# Autodesk Inventor assembly: base_body
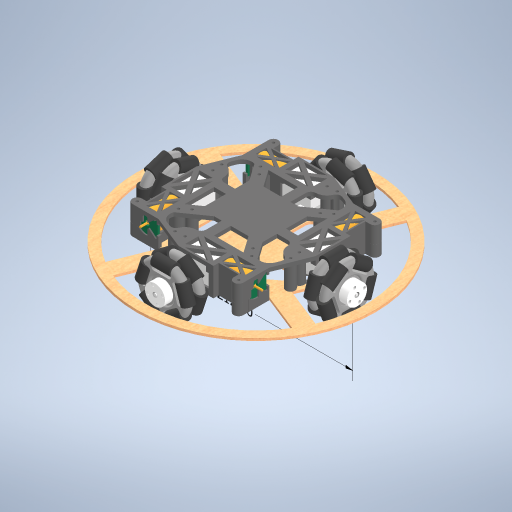
[picture p0: Inventor's stored thumbnail of the model, 512x512]
Saved by Autodesk Inventor 2024.1 (Build 281209000, 209)
## iProperties
Created: 2024-07-01
Part Number: base_body
Document SubType Name: Assembly
Designer: hibik
Author: hibik
## Documents named in this file (8)
- C:\Users\hibik\Desktop\ロボメカ\Rescue\2年\子機_本選\base_body.iam
- C:\Users\hibik\Desktop\ロボメカ\Rescue\2年\子機_本選\body_upper.ipt
- C:\Users\hibik\Desktop\ロボメカ\Rescue\2年\子機_本選\Motor.ipt
- C:\Users\hibik\Desktop\ロボメカ\Rescue\2年\子機_本選\encoder.ipt
- C:\Users\hibik\Desktop\ロボメカ\Rescue\2年\子機_本選\Motor_400.ipt
- C:\Users\hibik\Desktop\ロボメカ\Rescue\2年\子機_本選\オムニホイール.iam
- C:\Users\hibik\Desktop\ロボメカ\Rescue\2年\子機_本選\body_under.ipt
- C:\Users\hibik\Desktop\ロボメカ\Rescue\2年\子機_本選\plate.ipt
## Components (22 placed, 7 different names)
1. body_upper:1 — メイト:1, メイト:2, メイト:3, メイト:4, メイト:5, メイト:6, メイト:7, メイト:8, メイト:9, メイト:10, メイト:11, メイト:12, 挿入:1, 挿入:2, 挿入:3, 挿入:4, 角度:1, 角度:2, 角度:3, 角度:4, 挿入:5, 角度:5, 挿入:6, 角度:6, 挿入:7, 角度:7, 挿入:8, 角度:8, メイト:13, メイト:14, メイト:15, メイト:16, メイト:17, フラッシュ:1, フラッシュ:2
2. Motor:1 — メイト:1, メイト:9, メイト:10, 回転:1
3. Motor:2 — メイト:2, メイト:7, メイト:8, 回転:4
4. Motor:3 — メイト:4, メイト:5, メイト:6, 回転:3
5. Motor:4 — メイト:3, メイト:11, メイト:12, 回転:2
6. encoder:1 — 挿入:1, 角度:2
7. encoder:2 — 挿入:4, 角度:1
8. encoder:3 — 挿入:3, 角度:4
9. encoder:4 — 挿入:2, 角度:3
10. Motor_400:1 — 挿入:5, 角度:5, 挿入:11
11. Motor_400:2 — 挿入:6, 角度:6, 挿入:12
12. Motor_400:3 — 挿入:7, 角度:7, 挿入:9
13. Motor_400:4 — 挿入:8, 角度:8, 挿入:10
14. オムニホイール:1 [sub-assembly] — 回転:3
15. オムニホイール:2 [sub-assembly] — 回転:4
16. オムニホイール:3 [sub-assembly] — 回転:2
17. オムニホイール:4 [sub-assembly] — 回転:1
18. body_under:1 — 挿入:9, メイト:13
19. body_under:2 — 挿入:12, メイト:16
20. body_under:3 — 挿入:11, メイト:15
21. body_under:4 — 挿入:10, メイト:14
22. plate:1 — メイト:17, フラッシュ:1, フラッシュ:2
## Relationships (43: Mate 17, Insert 12, Angle 8, RevoluteJoint 4, Flush 2)
- メイト:1 [Mate]: body_upper:1 ↔ Motor:1
- メイト:2 [Mate]: body_upper:1 ↔ Motor:2
- メイト:3 [Mate]: body_upper:1 ↔ Motor:4
- メイト:4 [Mate]: body_upper:1 ↔ Motor:3
- メイト:5 [Mate]: body_upper:1 ↔ Motor:3
- メイト:6 [Mate]: body_upper:1 ↔ Motor:3
- メイト:7 [Mate]: body_upper:1 ↔ Motor:2
- メイト:8 [Mate]: body_upper:1 ↔ Motor:2
- メイト:9 [Mate]: body_upper:1 ↔ Motor:1
- メイト:10 [Mate]: body_upper:1 ↔ Motor:1
- メイト:11 [Mate]: body_upper:1 ↔ Motor:4
- メイト:12 [Mate]: body_upper:1 ↔ Motor:4
- 挿入:1 [Insert]: body_upper:1 ↔ encoder:1
- 挿入:2 [Insert]: body_upper:1 ↔ encoder:4
- 挿入:3 [Insert]: body_upper:1 ↔ encoder:3
- 挿入:4 [Insert]: body_upper:1 ↔ encoder:2
- 角度:1 [Angle] (0 deg): body_upper:1 ↔ encoder:2
- 角度:2 [Angle] (0 deg): body_upper:1 ↔ encoder:1
- 角度:3 [Angle] (0 deg): body_upper:1 ↔ encoder:4
- 角度:4 [Angle] (0 deg): body_upper:1 ↔ encoder:3
- 挿入:5 [Insert]: body_upper:1 ↔ Motor_400:1
- 角度:5 [Angle] (0 deg): body_upper:1 ↔ Motor_400:1
- 挿入:6 [Insert]: body_upper:1 ↔ Motor_400:2
- 角度:6 [Angle] (0 deg): body_upper:1 ↔ Motor_400:2
- 挿入:7 [Insert]: body_upper:1 ↔ Motor_400:3
- 角度:7 [Angle] (0 deg): body_upper:1 ↔ Motor_400:3
- 挿入:8 [Insert]: body_upper:1 ↔ Motor_400:4
- 角度:8 [Angle] (0 deg): body_upper:1 ↔ Motor_400:4
- 回転:1 [RevoluteJoint]: Motor:1 ↔ オムニホイール:4
- 回転:2 [RevoluteJoint]: Motor:4 ↔ オムニホイール:3
- 回転:3 [RevoluteJoint]: Motor:3 ↔ オムニホイール:1
- 回転:4 [RevoluteJoint]: Motor:2 ↔ オムニホイール:2
- 挿入:9 [Insert]: Motor_400:3 ↔ body_under:1
- メイト:13 [Mate]: body_upper:1 ↔ body_under:1
- 挿入:10 [Insert]: Motor_400:4 ↔ body_under:4
- 挿入:11 [Insert]: Motor_400:1 ↔ body_under:3
- 挿入:12 [Insert]: Motor_400:2 ↔ body_under:2
- メイト:14 [Mate]: body_upper:1 ↔ body_under:4
- メイト:15 [Mate]: body_upper:1 ↔ body_under:3
- メイト:16 [Mate]: body_upper:1 ↔ body_under:2
- メイト:17 [Mate]: body_upper:1 ↔ plate:1
- フラッシュ:1 [Flush]: body_upper:1 ↔ plate:1
- フラッシュ:2 [Flush]: body_upper:1 ↔ plate:1
